# Autodesk Inventor assembly: ferramenta
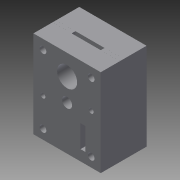
[picture p0: Inventor's stored thumbnail of the model, 180x180]
Saved by Autodesk Inventor 2015 (Build 190159000, 159)
## iProperties
Created: 2015-11-06
Part Number: ferramenta
Document SubType Name: Assembly
Designer: EriveltonDell
Author: EriveltonDell
## Documents named in this file (5)
- C:\Users\EriveltonDell\Documents\Centro Universitário da FEI\8 ciclo\Elementos de Máquina II\Projeto\Estampo\Desenho\ferramenta.iam
- C:\Users\EriveltonDell\Documents\Centro Universitário da FEI\8 ciclo\Elementos de Máquina II\Projeto\Estampo\Desenho\Matriz.ipt
- C:\Users\EriveltonDell\Documents\Centro Universitário da FEI\8 ciclo\Elementos de Máquina II\Projeto\Estampo\Desenho\regua guia 1.ipt
- C:\Users\EriveltonDell\Documents\Centro Universitário da FEI\8 ciclo\Elementos de Máquina II\Projeto\Estampo\Desenho\regua guia 2.ipt
- C:\Users\EriveltonDell\Documents\Centro Universitário da FEI\8 ciclo\Elementos de Máquina II\Projeto\Estampo\Desenho\Guia.ipt
## Components (4 placed, 4 different names)
1. Matriz:1 — Flush:1, Insert:1, Flush:2, Insert:2, Flush:3, Flush:4
2. regua guia 1:1 — Flush:1, Insert:1
3. regua guia 2:1 — Flush:2, Insert:2, Mate:1
4. Guia:1 — Flush:3, Flush:4, Mate:1
## Relationships (7: Flush 4, Insert 2, Mate 1)
- Flush:1: Matriz:1 ↔ regua guia 1:1
- Insert:1: Matriz:1 ↔ regua guia 1:1
- Flush:2: Matriz:1 ↔ regua guia 2:1
- Insert:2: Matriz:1 ↔ regua guia 2:1
- Flush:3: Matriz:1 ↔ Guia:1
- Flush:4: Matriz:1 ↔ Guia:1
- Mate:1: regua guia 2:1 ↔ Guia:1
